# Autodesk Inventor assembly: Viaduct_HorizontalSingle
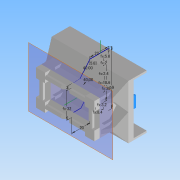
[picture p0: Inventor's stored thumbnail of the model, 180x180]
Saved by Autodesk Inventor 2021 (Build 250183000, 183)
## iProperties
Created: 2021-03-16
Part Number: Viaduct_HorizontalSingle
Document SubType Name: Assembly
Designer: kumagai
Author: kumagai
## Documents named in this file (6)
- Z:\Develop\CAD\PlaRails\ViaductPillarUnit\Viaduct_HorizontalSingle.iam
- Z:\Develop\CAD\PlaRails\ViaductPillarUnit\Viaduct_HorizontalSingle.ipt
- Z:\Develop\CAD\PlaRails\ViaductPillarUnit\VPU_EdgeBottom.ipt
- Z:\Develop\CAD\PlaRails\GlobalParameter.ipt
- Z:\Develop\CAD\PlaRails\RailJointFemale_filled.ipt
- Z:\Develop\CAD\PlaRails\RailJointMale_filled.ipt
## Components (5 placed, 4 different names)
1. Viaduct_HorizontalSingle:1 — メイト:2, フラッシュ:3, フラッシュ:4, メイト:3, メイト:4, メイト:5, メイト:6, フラッシュ:5, フラッシュ:6
2. VPU_EdgeBottom:1 — メイト:1, フラッシュ:1, フラッシュ:2, フラッシュ:3, フラッシュ:4
3. VPU_EdgeBottom:2 — メイト:1, フラッシュ:1, フラッシュ:2, メイト:2
4. RailJointFemale_filled:1 — メイト:4, メイト:5, フラッシュ:5
5. RailJointMale_filled:1 — メイト:3, メイト:6, フラッシュ:6
## Relationships (12: Mate 6, Flush 6)
- メイト:1 [Mate]: VPU_EdgeBottom:1 ↔ VPU_EdgeBottom:2
- フラッシュ:1 [Flush]: VPU_EdgeBottom:1 ↔ VPU_EdgeBottom:2
- フラッシュ:2 [Flush]: VPU_EdgeBottom:1 ↔ VPU_EdgeBottom:2
- メイト:2 [Mate] (-33 mm): Viaduct_HorizontalSingle:1 ↔ VPU_EdgeBottom:2
- フラッシュ:3 [Flush]: Viaduct_HorizontalSingle:1 ↔ VPU_EdgeBottom:1
- フラッシュ:4 [Flush]: Viaduct_HorizontalSingle:1 ↔ VPU_EdgeBottom:1
- メイト:3 [Mate]: Viaduct_HorizontalSingle:1 ↔ RailJointMale_filled:1
- メイト:4 [Mate]: Viaduct_HorizontalSingle:1 ↔ RailJointFemale_filled:1
- メイト:5 [Mate]: Viaduct_HorizontalSingle:1 ↔ RailJointFemale_filled:1
- メイト:6 [Mate]: Viaduct_HorizontalSingle:1 ↔ RailJointMale_filled:1
- フラッシュ:5 [Flush]: Viaduct_HorizontalSingle:1 ↔ RailJointFemale_filled:1
- フラッシュ:6 [Flush]: Viaduct_HorizontalSingle:1 ↔ RailJointMale_filled:1
## Named parameters: StraightLength = 215 mm, ViaductHeight = 66 mm
